# Autodesk Inventor assembly: akf-100-window
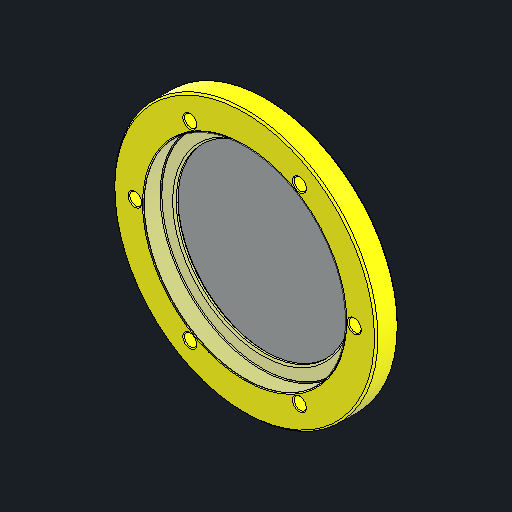
[picture p0: Inventor's stored thumbnail of the model, 512x512]
Saved by Autodesk Inventor 2026 (Build 300175050, 175E)
## iProperties
Created: 2025-12-12
Part Number: akf-100-window
Document SubType Name: Assembly
Designer: kuzmin
Author: kuzmin
## Documents named in this file (3)
- C:\Users\queezz\Dropbox\Drawings\PIHTI\PLD\akf-100-window.iam
- C:\Users\queezz\Dropbox\Drawings\PIHTI\PLD\glass-115-10.ipt
- C:\Users\queezz\Dropbox\Drawings\PIHTI\PLD\akf-100-window.ipt
## Components (2 placed, 2 different names)
1. glass-115-10:1
2. akf-100-window:1
## Relationships (1: WeldJoint 1)
- [WeldJoint]: glass-115-10:1 ↔ akf-100-window:1
